# Autodesk Inventor assembly: Feeder
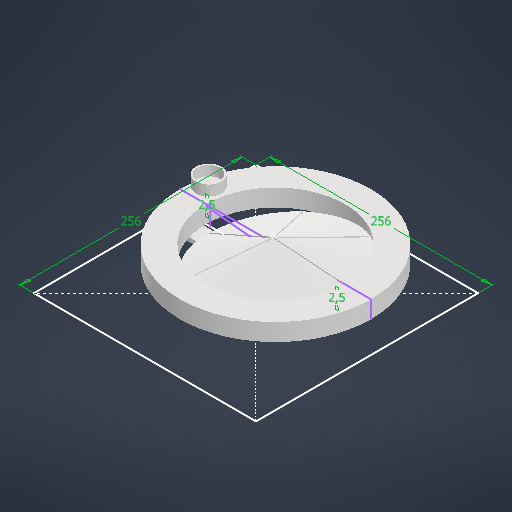
[picture p0: Inventor's stored thumbnail of the model, 512x512]
Saved by Autodesk Inventor 2026 (Build 300175050, 175E)
## iProperties
Created: 2026-03-25
Part Number: Feeder
Document SubType Name: Assembly
Designer: sniel
Author: sniel
## Documents named in this file (6)
- C:\Users\sniel\OneDrive\SDU\4. Semester\Applied automation\feeder\Feeder.iam
- C:\Users\sniel\OneDrive\SDU\4. Semester\Applied automation\feeder\Bottle.ipt
- C:\Users\sniel\OneDrive\SDU\4. Semester\Applied automation\feeder\base plate.ipt
- C:\Users\sniel\OneDrive\SDU\4. Semester\Applied automation\feeder\central disk.ipt
- C:\Users\sniel\OneDrive\SDU\4. Semester\Applied automation\feeder\outerspinner.ipt
- C:\Users\sniel\OneDrive\SDU\4. Semester\Applied automation\feeder\base mount for central centrifuge.ipt
## Components (5 placed, 5 different names)
1. Bottle:1
2. base plate:1
3. central disk:1 — Mate:1
4. outerspinner:1
5. base mount for central centrifuge:1 — Mate:1
## Relationships (1: Mate 1)
- Mate:1: central disk:1 ↔ base mount for central centrifuge:1
